# Autodesk Inventor assembly: MainAssembly
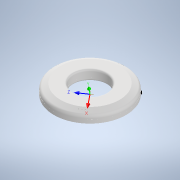
[picture p0: Inventor's stored thumbnail of the model, 180x180]
Saved by Autodesk Inventor 2020.2 (Build 242310000, 310)
## iProperties
Created: 2022-04-27
Part Number: MainAssembly
Document SubType Name: Assembly
Designer: Mitch
Author: Mitch
## Documents named in this file (8)
- E:\Youtube Channel\Pojects\Keg Manager\MainAssembly.iam
- E:\Youtube Channel\Pojects\Keg Manager\Bottom.ipt
- E:\Youtube Channel\Pojects\Keg Manager\Top.ipt
- E:\Youtube Channel\Pojects\Keg Manager\Keg.ipt
- E:\Youtube Channel\Pojects\Keg Manager\50-kg-load-cell-resistance-strain-half-bridge-sensor-1.snapshot.2\50 kg Load Cell Resistance Strain Half Bridge Sensor.iam
- E:\Youtube Channel\Pojects\Keg Manager\Feet.ipt
- E:\Youtube Channel\Pojects\Keg Manager\Feet Cap.ipt
- E:\Youtube Channel\Pojects\Keg Manager\DC Jack\DC Jack Panel Mount Base.ipt
## Components (16 placed, 7 different names)
1. Bottom:1 — Mate:1, Mate:2, Tangent:1, Mate:25
2. Top:1 — Mate:1, Mate:2, Mate:3, Mate:4, Flush:1, Flush:2, Flush:3, Flush:4, Mate:5, Mate:6, Mate:7, Mate:8
3. Keg:1 — Mate:3, Mate:4
4. 50 kg Load Cell Resistance Strain Half Bridge Sensor:1 [sub-assembly] — Flush:1, Mate:5, Mate:11, Mate:15
5. 50 kg Load Cell Resistance Strain Half Bridge Sensor:2 [sub-assembly] — Flush:2, Mate:8, Mate:9, Mate:10
6. 50 kg Load Cell Resistance Strain Half Bridge Sensor:3 [sub-assembly] — Flush:4, Mate:6, Mate:12, Mate:14
7. 50 kg Load Cell Resistance Strain Half Bridge Sensor:4 [sub-assembly] — Flush:3, Mate:7, Mate:13, Mate:16
8. Feet:1 — Mate:17, Mate:18
9. Feet:2 — Mate:19, Mate:20
10. Feet:3 — Mate:21, Mate:22
11. Feet:4 — Mate:23, Mate:24
12. Feet Cap:1 — Mate:9, Mate:10, Mate:17, Mate:18
13. Feet Cap:2 — Mate:11, Mate:15, Mate:19, Mate:20
14. Feet Cap:3 — Mate:12, Mate:14, Mate:21, Mate:22
15. Feet Cap:4 — Mate:13, Mate:16, Mate:23, Mate:24
16. DC Jack Panel Mount Base:1 — Tangent:1, Mate:25
## Relationships (30: Mate 25, Flush 4, Tangent 1)
- Mate:1: Bottom:1 ↔ Top:1
- Mate:2: Bottom:1 ↔ Top:1
- Mate:3: Top:1 ↔ Keg:1
- Mate:4: Top:1 ↔ Keg:1
- Flush:1: Top:1 ↔ 50 kg Load Cell Resistance Strain Half Bridge Sensor:1
- Flush:2: Top:1 ↔ 50 kg Load Cell Resistance Strain Half Bridge Sensor:2
- Flush:3: Top:1 ↔ 50 kg Load Cell Resistance Strain Half Bridge Sensor:4
- Flush:4: Top:1 ↔ 50 kg Load Cell Resistance Strain Half Bridge Sensor:3
- Mate:5: Top:1 ↔ 50 kg Load Cell Resistance Strain Half Bridge Sensor:1
- Mate:6: Top:1 ↔ 50 kg Load Cell Resistance Strain Half Bridge Sensor:3
- Mate:7: Top:1 ↔ 50 kg Load Cell Resistance Strain Half Bridge Sensor:4
- Mate:8: Top:1 ↔ 50 kg Load Cell Resistance Strain Half Bridge Sensor:2
- Mate:9: 50 kg Load Cell Resistance Strain Half Bridge Sensor:2 ↔ Feet Cap:1
- Mate:10: 50 kg Load Cell Resistance Strain Half Bridge Sensor:2 ↔ Feet Cap:1
- Mate:11: 50 kg Load Cell Resistance Strain Half Bridge Sensor:1 ↔ Feet Cap:2
- Mate:12: 50 kg Load Cell Resistance Strain Half Bridge Sensor:3 ↔ Feet Cap:3
- Mate:13: 50 kg Load Cell Resistance Strain Half Bridge Sensor:4 ↔ Feet Cap:4
- Mate:14: 50 kg Load Cell Resistance Strain Half Bridge Sensor:3 ↔ Feet Cap:3
- Mate:15: 50 kg Load Cell Resistance Strain Half Bridge Sensor:1 ↔ Feet Cap:2
- Mate:16: 50 kg Load Cell Resistance Strain Half Bridge Sensor:4 ↔ Feet Cap:4
- Mate:17: Feet:1 ↔ Feet Cap:1
- Mate:18: Feet:1 ↔ Feet Cap:1
- Mate:19: Feet:2 ↔ Feet Cap:2
- Mate:20: Feet:2 ↔ Feet Cap:2
- Mate:21: Feet:3 ↔ Feet Cap:3
- Mate:22: Feet:3 ↔ Feet Cap:3
- Mate:23: Feet:4 ↔ Feet Cap:4
- Mate:24: Feet:4 ↔ Feet Cap:4
- Tangent:1: Bottom:1 ↔ DC Jack Panel Mount Base:1
- Mate:25: Bottom:1 ↔ DC Jack Panel Mount Base:1
